# Autodesk Inventor assembly: Shoulder Joint Assembly
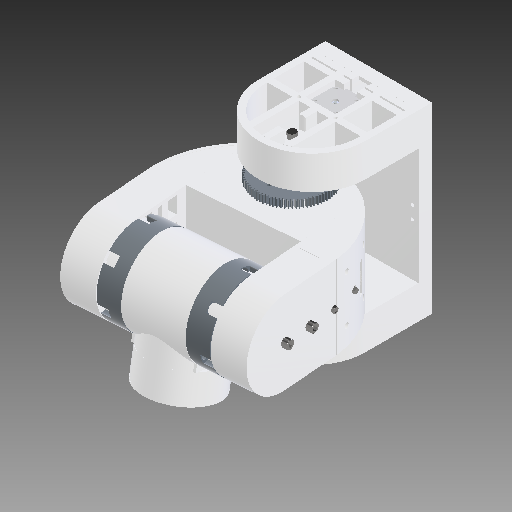
[picture p0: Inventor's stored thumbnail of the model, 512x512]
Saved by Autodesk Inventor 2017 SP1 (Build 210196100, 196)
## iProperties
Created: 2017-06-01
Part Number: Shoulder Joint Assembly
Document SubType Name: Assembly
Designer: Zach
Author: Zach
## Documents named in this file (25)
- C:\Users\Zach\Documents\GitHub\tr1\src\Body\Arm Assembly\Shoulder Joint Assembly\Shoulder Joint Assembly.iam
- C:\Users\Zach\Documents\GitHub\tr1\src\Body\Arm Assembly\Shoulder Joint Assembly\SJ002.ipt
- C:\Users\Zach\Documents\GitHub\tr1\src\Body\Arm Assembly\Shoulder Joint Assembly\SJ003.ipt
- C:\Users\Zach\Documents\GitHub\tr1\src\Body\Arm Assembly\Shoulder Joint Assembly\SJ001.ipt
- C:\Users\Zach\Documents\GitHub\tr1\lib\Stepper Motor - NEMA 17\NEMA17.ipt
- C:\Users\Zach\Documents\GitHub\tr1\src\Body\Arm Assembly\Shoulder Joint Assembly\SJ004.ipt
- C:\Users\Zach\Documents\GitHub\tr1\src\Body\Arm Assembly\Shoulder Joint Assembly\SJ005.ipt
- C:\Users\Zach\Documents\GitHub\tr1\src\Body\Arm Assembly\Shoulder Joint Assembly\SJ006.ipt
- C:\Users\Zach\Documents\GitHub\tr1\lib\U51105\U51105.ipt
- C:\Users\Zach\Documents\GitHub\tr1\lib\6201RS\6201RS.ipt
- C:\Users\Zach\Documents\GitHub\tr1\src\Body\Arm Assembly\Shoulder Joint Assembly\SJ007.ipt
- C:\Users\Zach\Documents\GitHub\tr1\src\Body\Arm Assembly\Shoulder Joint Assembly\SJ008.ipt
- C:\Users\Zach\Documents\GitHub\tr1\src\Body\Arm Assembly\Shoulder Joint Assembly\Shoulder Joint Assembly\Design Accelerator\Spur Gears1.iam
- C:\Users\Zach\Documents\GitHub\tr1\src\Body\Arm Assembly\Shoulder Joint Assembly\SJ009.ipt
- C:\Users\Zach\Documents\GitHub\tr1\lib\22x8x8mm Bearing.ipt
- C:\Users\Zach\Documents\GitHub\tr1\src\Body\Arm Assembly\Shoulder Joint Assembly\Shoulder Joint Assembly\Design Accelerator\Spur Gears3.iam
- C:\Users\Zach\Documents\GitHub\tr1\src\Body\Arm Assembly\Shoulder Joint Assembly\Shoulder Joint Assembly\Design Accelerator\Spur Gears4.iam
- C:\Users\Zach\Documents\GitHub\tr1\src\Body\Arm Assembly\Shoulder Joint Assembly\SJ018.ipt
- C:\Users\Zach\Documents\GitHub\tr1\lib\Stepper Motor - NEMA 24\StepperMotor_Nema24.iam
- C:\Users\Zach\Documents\Inventor\Content Center Files\R2017\en-US\IS 2269\IS 2269 - M8 x 30.ipt
- C:\Users\Zach\Documents\Inventor\Content Center Files\R2017\en-US\ISO 4015\ISO 4015 - M5 x 25.ipt
- C:\Users\Zach\Documents\GitHub\tr1\src\Body\Arm Assembly\Shoulder Joint Assembly\Shoulder Joint Assembly\Design Accelerator\Spur Gears5.iam
- C:\Users\Zach\Documents\GitHub\tr1\src\Body\Arm Assembly\Shoulder Joint Assembly\SJ019.ipt
- C:\Users\Zach\Documents\GitHub\tr1\lib\QS12MM250\QS12MM250.ipt
- C:\Users\Zach\Documents\GitHub\tr1\lib\Gearbox 128;1\Gearbox 128;1.iam
## Components (40 placed, 21 different names)
1. SJ001:1 — Mate:47, Mate:325, Mate:326, Mate:330, Mate:331, Mate:332, Mate:333, Mate:352, Mate:353, Mate:354
2. SJ001:2 — Mate:302, Mate:303, Mate:304, Mate:306, Mate:307, Mate:308, Mate:309, Mate:310, Mate:311, Mate:312, Mate:313, Mate:322, Mate:324, Mate:357
3. SJ002:1 — Mate:1, Mate:4, Mate:8, Mate:9, Mate:355, Mate:356
4. SJ002:2 — Mate:18, Mate:19, Mate:20, Mate:349, Mate:350, Mate:351
5. SJ003:1 — Mate:1, Mate:4, Mate:8, Mate:9, Mate:18, Mate:19, Mate:20, Mate:148, Mate:149, Mate:150, Mate:295, Mate:358, Mate:359, Mate:360
6. SJ004:1 — Mate:130, Mate:163, Mate:212, Mate:213, Mate:214, Mate:300, Mate:301, Mate:302, Mate:303, Mate:304, Mate:314, Mate:315, Mate:317, Mate:319, Mate:320
7. SJ004:2 — Mate:47, Mate:54, Mate:55, Mate:56, Mate:216, Mate:217, Mate:325, Mate:326, Mate:334, Mate:335
8. SJ005:1 — Mate:54, Mate:55, Mate:56, Mate:60, Mate:67, Mate:69, Mate:70, Flush:1, Mate:218, Mate:340, Mate:346
9. SJ005:2 — Mate:68, Mate:82, Mate:84, Mate:130, Mate:136, Flush:1, Mate:163, Mate:214, Mate:218, Mate:340
10. SJ006:2 — Mate:67, Mate:68, Mate:69, Mate:70, Mate:78, Mate:79, Mate:83
11. SJ007:1 — Mate:121, Mate:122, Mate:123, Mate:133, Mate:342, Mate:343
12. SJ007:2 — Mate:133, Mate:342, Mate:343, Mate:344, Mate:345
13. SJ008:2 — Mate:97, Mate:98, Mate:99, Mate:112, Mate:121, Mate:122, Mate:123, Mate:124, Mate:131
14. SJ009:1 — Mate:212, Mate:213
15. SJ009:2 — Mate:216, Mate:217
16. SJ018:1 — Mate:290, Mate:291, Mate:292
17. U51105:1 — Mate:131, Mate:139
18. U51105:2 — Mate:78, Mate:79
19. 6201RS:1 — Mate:82, Mate:138
20. 6201RS:2 — Mate:83, Mate:84
21. 22x8x8mm Bearing:4 — Mate:327, Flush:329
22. 22x8x8mm Bearing:5 — Mate:328, Mate:329
23. Spur Gears:1 [sub-assembly] — Mate:136, Mate:137, Mate:138, Mate:139
24. Spur Gears:3 [sub-assembly] — Mate:306, Mate:307, Mate:308, Mate:309, Mate:321, Mate:322, Mate:323, Mate:324, Mate:327, Flush:329, Mate:328, Mate:329
25. Spur Gears:6 [sub-assembly] — Mate:286, Mate:290, Mate:291, Mate:292, Mate:295
26. NEMA17:1 — Mate:148, Mate:149, Mate:150, Mate:286
27. NEMA17:2 — Mate:97, Mate:98, Mate:99, Mate:137
28. StepperMotor_Nema24:1 [sub-assembly] — Mate:300, Mate:301, Mate:316, Mate:320
29. IS 2269 M8 x 30:1 — Mate:310, Mate:311, Mate:321
30. IS 2269 M8 x 30:2 — Mate:312, Mate:313, Mate:323
31. ISO 4015 M5 x 25:1 — Mate:314, Mate:315, Mate:318
32. Spur Gears:7 [sub-assembly] — Mate:316, Mate:317, Mate:318, Mate:319
33. IS 2269 M8 x 30:3 — Mate:330, Mate:331
34. IS 2269 M8 x 30:4 — Mate:332, Mate:333
35. ISO 4015 M5 x 25:2 — Mate:334, Mate:335
36. SJ019:1 — Mate:344, Mate:345, Mate:346, Mate:347, Mate:348
37. QS12MM250:1 — Mate:347, Mate:348
38. Gearbox 128;1:1 [sub-assembly] — Mate:349, Mate:350, Mate:351, Mate:357
39. Gearbox 128;1:2 [sub-assembly] — Mate:352, Mate:353, Mate:354, Mate:355, Mate:356
40. Gearbox 128;1:3 [sub-assembly] — Mate:358, Mate:359, Mate:360
## Relationships (108: Mate 106, Flush 2)
- Mate:1: SJ002:1 ↔ SJ003:1
- Mate:4: SJ002:1 ↔ SJ003:1
- Mate:8: SJ002:1 ↔ SJ003:1
- Mate:9: SJ002:1 ↔ SJ003:1
- Mate:18: SJ002:2 ↔ SJ003:1
- Mate:19: SJ002:2 ↔ SJ003:1
- Mate:20: SJ002:2 ↔ SJ003:1
- Mate:47: SJ001:1 ↔ SJ004:2
- Mate:54: SJ004:2 ↔ SJ005:1
- Mate:55: SJ004:2 ↔ SJ005:1
- Mate:56: SJ004:2 ↔ SJ005:1
- Mate:60: SJ005:1
- Mate:67: SJ005:1 ↔ SJ006:2
- Mate:68: SJ005:2 ↔ SJ006:2
- Mate:69: SJ005:1 ↔ SJ006:2
- Mate:70: SJ005:1 ↔ SJ006:2
- Mate:78: SJ006:2 ↔ U51105:2
- Mate:79: SJ006:2 ↔ U51105:2
- Mate:82: SJ005:2 ↔ 6201RS:1
- Mate:83: SJ006:2 ↔ 6201RS:2
- Mate:84: SJ005:2 ↔ 6201RS:2
- Mate:97: SJ008:2 ↔ NEMA17:2
- Mate:98: SJ008:2 ↔ NEMA17:2
- Mate:99: SJ008:2 ↔ NEMA17:2
- Mate:112: SJ008:2
- Mate:121: SJ007:1 ↔ SJ008:2
- Mate:122: SJ007:1 ↔ SJ008:2
- Mate:123: SJ007:1 ↔ SJ008:2
- Mate:124: SJ008:2
- Mate:130: SJ004:1 ↔ SJ005:2
- Mate:131: SJ008:2 ↔ U51105:1
- Mate:133: SJ007:1 ↔ SJ007:2
- Mate:136: SJ005:2 ↔ Spur Gears:1
- Mate:137: Spur Gears:1 ↔ NEMA17:2
- Mate:138: 6201RS:1 ↔ Spur Gears:1
- Mate:139: U51105:1 ↔ Spur Gears:1
- Mate:148: SJ003:1 ↔ NEMA17:1
- Mate:149: SJ003:1 ↔ NEMA17:1
- Mate:150: SJ003:1 ↔ NEMA17:1
- Flush:1: SJ005:1 ↔ SJ005:2
- Mate:163: SJ004:1 ↔ SJ005:2
- Mate:212: SJ004:1 ↔ SJ009:1
- Mate:213: SJ004:1 ↔ SJ009:1
- Mate:214: SJ004:1 ↔ SJ005:2
- Mate:216: SJ004:2 ↔ SJ009:2
- Mate:217: SJ004:2 ↔ SJ009:2
- Mate:218: SJ005:1 ↔ SJ005:2
- Mate:286: Spur Gears:6 ↔ NEMA17:1
- Mate:290: SJ018:1 ↔ Spur Gears:6
- Mate:291: SJ018:1 ↔ Spur Gears:6
- Mate:292: SJ018:1 ↔ Spur Gears:6
- Mate:295: SJ003:1 ↔ Spur Gears:6
- Mate:300: SJ004:1 ↔ StepperMotor_Nema24:1
- Mate:301: SJ004:1 ↔ StepperMotor_Nema24:1
- Mate:302: SJ001:2 ↔ SJ004:1
- Mate:303: SJ001:2 ↔ SJ004:1
- Mate:304: SJ001:2 ↔ SJ004:1
- Mate:306: SJ001:2 ↔ Spur Gears:3
- Mate:307: SJ001:2 ↔ Spur Gears:3
- Mate:308: SJ001:2 ↔ Spur Gears:3
- Mate:309: SJ001:2 ↔ Spur Gears:3
- Mate:310: SJ001:2 ↔ IS 2269 M8 x 30:1
- Mate:311: SJ001:2 ↔ IS 2269 M8 x 30:1
- Mate:312: SJ001:2 ↔ IS 2269 M8 x 30:2
- Mate:313: SJ001:2 ↔ IS 2269 M8 x 30:2
- Mate:314: SJ004:1 ↔ ISO 4015 M5 x 25:1
- Mate:315: SJ004:1 ↔ ISO 4015 M5 x 25:1
- Mate:316: StepperMotor_Nema24:1 ↔ Spur Gears:7
- Mate:317: SJ004:1 ↔ Spur Gears:7
- Mate:318: ISO 4015 M5 x 25:1 ↔ Spur Gears:7
- Mate:319: SJ004:1 ↔ Spur Gears:7
- Mate:320: SJ004:1 ↔ StepperMotor_Nema24:1
- Mate:321: Spur Gears:3 ↔ IS 2269 M8 x 30:1
- Mate:322: SJ001:2 ↔ Spur Gears:3
- Mate:323: Spur Gears:3 ↔ IS 2269 M8 x 30:2
- Mate:324: SJ001:2 ↔ Spur Gears:3
- Mate:325: SJ001:1 ↔ SJ004:2
- Mate:326: SJ001:1 ↔ SJ004:2
- Mate:327: 22x8x8mm Bearing:4 ↔ Spur Gears:3
- Flush:329: 22x8x8mm Bearing:4 ↔ Spur Gears:3
- Mate:328: 22x8x8mm Bearing:5 ↔ Spur Gears:3
- Mate:329: 22x8x8mm Bearing:5 ↔ Spur Gears:3
- Mate:330: SJ001:1 ↔ IS 2269 M8 x 30:3
- Mate:331: SJ001:1 ↔ IS 2269 M8 x 30:3
- Mate:332: SJ001:1 ↔ IS 2269 M8 x 30:4
- Mate:333: SJ001:1 ↔ IS 2269 M8 x 30:4
- Mate:334: SJ004:2 ↔ ISO 4015 M5 x 25:2
- Mate:335: SJ004:2 ↔ ISO 4015 M5 x 25:2
- Mate:340: SJ005:1 ↔ SJ005:2
- Mate:342: SJ007:1 ↔ SJ007:2
- Mate:343: SJ007:1 ↔ SJ007:2
- Mate:344: SJ007:2 ↔ SJ019:1
- Mate:345: SJ007:2 ↔ SJ019:1
- Mate:346: SJ005:1 ↔ SJ019:1
- Mate:347: SJ019:1 ↔ QS12MM250:1
- Mate:348: SJ019:1 ↔ QS12MM250:1
- Mate:349: SJ002:2 ↔ Gearbox 128;1:1
- Mate:350: SJ002:2 ↔ Gearbox 128;1:1
- Mate:351: SJ002:2 ↔ Gearbox 128;1:1
- Mate:352: SJ001:1 ↔ Gearbox 128;1:2
- Mate:353: SJ001:1 ↔ Gearbox 128;1:2
- Mate:354: SJ001:1 ↔ Gearbox 128;1:2
- Mate:355: SJ002:1 ↔ Gearbox 128;1:2
- Mate:356: SJ002:1 ↔ Gearbox 128;1:2
- Mate:357: SJ001:2 ↔ Gearbox 128;1:1
- Mate:358: SJ003:1 ↔ Gearbox 128;1:3
- Mate:359: SJ003:1 ↔ Gearbox 128;1:3
- Mate:360: SJ003:1 ↔ Gearbox 128;1:3
